# Autodesk Inventor assembly: complete setup met relief
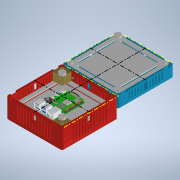
[picture p0: Inventor's stored thumbnail of the model, 180x180]
Saved by Autodesk Inventor 2021 (Build 250183000, 183)
## iProperties
Created: 2023-11-13
Part Number: complete setup met relief
Document SubType Name: Assembly
Designer: Elias
Author: Elias
## Documents named in this file (11)
- D:\Hoge school ICT\2.0 Project experience 2.1\Tekeningen\13_11_2023\complete setup met relief.iam
- D:\Hoge school ICT\2.0 Project experience 2.1\Tekeningen\13_11_2023\Led behuizing dubbele hoogte.ipt
- D:\Hoge school ICT\2.0 Project experience 2.1\Tekeningen\13_11_2023\Led deksel hub.ipt
- D:\Hoge school ICT\2.0 Project experience 2.1\Tekeningen\13_11_2023\ledstrip.ipt
- D:\Hoge school ICT\2.0 Project experience 2.1\Tekeningen\13_11_2023\Led behuizing.ipt
- D:\Hoge school ICT\2.0 Project experience 2.1\Tekeningen\13_11_2023\Led deksel hub zonder pi.ipt
- D:\Hoge school ICT\2.0 Project experience 2.1\Tekeningen\13_11_2023\Magneet.ipt
- D:\Hoge school ICT\2.0 Project experience 2.1\Tekeningen\13_11_2023\magneet stand-offs.ipt
- D:\Hoge school ICT\2.0 Project experience 2.1\Tekeningen\13_11_2023\Raspberry Pi 4 Model B.iam
- D:\Hoge school ICT\2.0 Project experience 2.1\Tekeningen\13_11_2023\spacer dubbele hoogte behuizing.ipt
- D:\Hoge school ICT\2.0 Project experience 2.1\Tekeningen\13_11_2023\magneet stand-offs16 mm.ipt
## Components (19 placed, 10 different names)
1. Led behuizing dubbele hoogte:1 — Mate:1, Mate:2, Mate:10, Flush:7, Flush:8, Mate:11, Mate:20, Mate:21, Flush:9, Mate:22, Mate:23, Flush:10
2. Led deksel hub:1 — Mate:1, Mate:2, Mate:3, Mate:4, Mate:5, Mate:6, Flush:2, Flush:3, Flush:4, Flush:5, Flush:6, Mate:11, Mate:17, Mate:18, Mate:19
3. ledstrip:1 — Mate:6, Flush:3, Flush:6, Mate:7
4. ledstrip:2 — Mate:5, Flush:2, Mate:7, Mate:8
5. ledstrip:3 — Mate:3, Flush:5, Mate:9
6. ledstrip:4 — Mate:4, Flush:4, Mate:8, Mate:9
7. Led behuizing:1 — Mate:10, Flush:7, Flush:8, Mate:12, Mate:13, Mate:14
8. Led deksel hub zonder pi:1 — Mate:12, Mate:13, Mate:14, Insert:1, Insert:3, Mate:16
9. magneet stand-offs:2 — Insert:1, Insert:4
10. magneet stand-offs:3 — Insert:3, Mate:15
11. Magneet:1 — Insert:4
12. Magneet:2 — Mate:15, Mate:16
13. Raspberry Pi 4 Model B:1 [sub-assembly] — Mate:17, Mate:18, Mate:19
14. spacer dubbele hoogte behuizing:1 — Mate:20, Mate:21, Flush:9, Mate:25, Flush:12, Mate:27
15. spacer dubbele hoogte behuizing:2 — Mate:22, Mate:23, Flush:10, Mate:24, Flush:11, Mate:29
16. magneet stand-offs16 mm:1 — Mate:24, Flush:11, Mate:28
17. magneet stand-offs16 mm:2 — Mate:25, Flush:12, Mate:26
18. Magneet:3 — Mate:26, Mate:27
19. Magneet:5 — Mate:28, Mate:29
## Relationships (43: Mate 29, Flush 11, Insert 3)
- Mate:1: Led behuizing dubbele hoogte:1 ↔ Led deksel hub:1
- Mate:2: Led behuizing dubbele hoogte:1 ↔ Led deksel hub:1
- Mate:3: Led deksel hub:1 ↔ ledstrip:3
- Mate:4: Led deksel hub:1 ↔ ledstrip:4
- Mate:5: Led deksel hub:1 ↔ ledstrip:2
- Mate:6: Led deksel hub:1 ↔ ledstrip:1
- Flush:2 (32 mm): Led deksel hub:1 ↔ ledstrip:2
- Flush:3 (32 mm): Led deksel hub:1 ↔ ledstrip:1
- Flush:4 (32 mm): Led deksel hub:1 ↔ ledstrip:4
- Flush:5 (32 mm): Led deksel hub:1 ↔ ledstrip:3
- Flush:6 (25 mm): Led deksel hub:1 ↔ ledstrip:1
- Mate:7 (20 mm): ledstrip:1 ↔ ledstrip:2
- Mate:8 (20 mm): ledstrip:2 ↔ ledstrip:4
- Mate:9 (20 mm): ledstrip:3 ↔ ledstrip:4
- Mate:10: Led behuizing dubbele hoogte:1 ↔ Led behuizing:1
- Flush:7: Led behuizing dubbele hoogte:1 ↔ Led behuizing:1
- Flush:8: Led behuizing dubbele hoogte:1 ↔ Led behuizing:1
- Mate:11: Led behuizing dubbele hoogte:1 ↔ Led deksel hub:1
- Mate:12: Led behuizing:1 ↔ Led deksel hub zonder pi:1
- Mate:13: Led behuizing:1 ↔ Led deksel hub zonder pi:1
- Mate:14: Led behuizing:1 ↔ Led deksel hub zonder pi:1
- Insert:1: Led deksel hub zonder pi:1 ↔ magneet stand-offs:2
- Insert:3: Led deksel hub zonder pi:1 ↔ magneet stand-offs:3
- Insert:4 (-9 mm): magneet stand-offs:2 ↔ Magneet:1
- Mate:15: magneet stand-offs:3 ↔ Magneet:2
- Mate:16: Led deksel hub zonder pi:1 ↔ Magneet:2
- Mate:17: Led deksel hub:1 ↔ Raspberry Pi 4 Model B:1
- Mate:18: Led deksel hub:1 ↔ Raspberry Pi 4 Model B:1
- Mate:19: Led deksel hub:1 ↔ Raspberry Pi 4 Model B:1
- Mate:20: Led behuizing dubbele hoogte:1 ↔ spacer dubbele hoogte behuizing:1
- Mate:21: Led behuizing dubbele hoogte:1 ↔ spacer dubbele hoogte behuizing:1
- Flush:9: Led behuizing dubbele hoogte:1 ↔ spacer dubbele hoogte behuizing:1
- Mate:22: Led behuizing dubbele hoogte:1 ↔ spacer dubbele hoogte behuizing:2
- Mate:23: Led behuizing dubbele hoogte:1 ↔ spacer dubbele hoogte behuizing:2
- Flush:10: Led behuizing dubbele hoogte:1 ↔ spacer dubbele hoogte behuizing:2
- Mate:24: spacer dubbele hoogte behuizing:2 ↔ magneet stand-offs16 mm:1
- Flush:11: spacer dubbele hoogte behuizing:2 ↔ magneet stand-offs16 mm:1
- Mate:25: spacer dubbele hoogte behuizing:1 ↔ magneet stand-offs16 mm:2
- Flush:12: spacer dubbele hoogte behuizing:1 ↔ magneet stand-offs16 mm:2
- Mate:26: magneet stand-offs16 mm:2 ↔ Magneet:3
- Mate:27: spacer dubbele hoogte behuizing:1 ↔ Magneet:3
- Mate:28: magneet stand-offs16 mm:1 ↔ Magneet:5
- Mate:29: spacer dubbele hoogte behuizing:2 ↔ Magneet:5
